# Autodesk Inventor assembly: Core
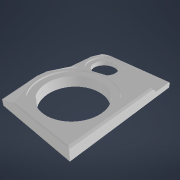
[picture p0: Inventor's stored thumbnail of the model, 180x180]
Saved by Autodesk Inventor 2022 (Build 260153000, 153)
## iProperties
Created: 2022-04-08
Part Number: Core
Document SubType Name: Assembly
Designer: Kalugin_a
Author: Kalugin_a
## Documents named in this file (3)
- D:\GitHUB\MELAS\Workspace\BoordyaBeatBox\Core.iam
- D:\GitHUB\MELAS\Workspace\BoordyaBeatBox\Front_L.ipt
- D:\GitHUB\MELAS\Workspace\BoordyaBeatBox\Front1.ipt
## Components (2 placed, 2 different names)
1. Front_L:1 — Совмещение:1, Совмещение:2
2. Front1:1 — Совмещение:1, Совмещение:2
## Relationships (2: Mate 2)
- Совмещение:1 [Mate]: Front_L:1 ↔ Front1:1
- Совмещение:2 [Mate]: Front_L:1 ↔ Front1:1
